# Autodesk Inventor assembly: Product
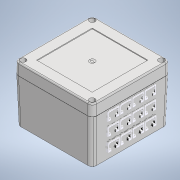
[picture p0: Inventor's stored thumbnail of the model, 180x180]
Saved by Autodesk Inventor 2021 (Build 250183000, 183)
## iProperties
Created: 2023-08-06
Part Number: Product
Document SubType Name: Assembly
Designer: michal
Author: michal
## Documents named in this file (3)
- C:\Users\micha\OneDrive\Dokumenty\GitHub\escape_room_hw_v2\Enclosure\Product.iam
- C:\Users\micha\OneDrive\Dokumenty\GitHub\escape_room_hw_v2\Enclosure\Commercial\139344992-9-zp105_105_75jph_tm\zp105_105_75jph_tm.iam
- C:\Users\micha\OneDrive\Dokumenty\GitHub\escape_room_hw_v2\Enclosure\Commercial\pcb stack.iam
## Components (2 placed, 2 different names)
1. zp105_105_75jph_tm:1 [sub-assembly] — Mate:1, Mate:2, Mate:3
2. pcb stack:1 [sub-assembly] — Mate:1, Mate:2, Mate:3
## Relationships (3: Mate 3)
- Mate:1: zp105_105_75jph_tm:1 ↔ pcb stack:1
- Mate:2: zp105_105_75jph_tm:1 ↔ pcb stack:1
- Mate:3: zp105_105_75jph_tm:1 ↔ pcb stack:1
